# Autodesk Inventor assembly: Ensamble
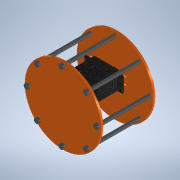
[picture p0: Inventor's stored thumbnail of the model, 180x180]
Saved by Autodesk Inventor 2021 (Build 250183000, 183)
## iProperties
Created: 2021-04-02
Part Number: Ensamble
Document SubType Name: Assembly
Designer: diego
Author: diego
## Documents named in this file (5)
- C:\Users\diego\Desktop\Diego\Utadeo 2021-1\Robotica Industrial\Corte 2\Solido planos\Ensamble.iam
- C:\Users\diego\Desktop\Diego\Utadeo 2021-1\Robotica Industrial\Corte 2\Solido planos\Base3.ipt
- C:\Users\diego\Desktop\Diego\Utadeo 2021-1\Robotica Industrial\Corte 2\Solido planos\Tornillo.ipt
- C:\Users\diego\Desktop\Diego\Utadeo 2021-1\Robotica Industrial\Corte 2\Solido planos\Servo.ipt
- C:\Users\diego\Desktop\Diego\Utadeo 2021-1\Robotica Industrial\Corte 2\Solido planos\Base1.iam
## Components (11 placed, 4 different names)
1. Base3:1 — Rígido:1, Rígido:2, Rígido:3, Rígido:4, Rígido:5, Rígido:6, Rígido:7, Rígido:8
2. Tornillo:1 — Rígido:1
3. Tornillo:2 — Rígido:2, Rígido:9
4. Tornillo:3 — Rígido:3
5. Tornillo:4 — Rígido:4
6. Tornillo:5 — Rígido:5
7. Tornillo:6 — Rígido:6
8. Tornillo:7 — Rígido:7
9. Tornillo:8 — Rígido:8
10. Servo:1 — Coincidencia:1
11. Base1:1 [sub-assembly] — Rígido:9, Coincidencia:1
## Relationships (10: WeldJoint 9, Mate 1)
- Rígido:1 [WeldJoint]: Base3:1 ↔ Tornillo:1
- Rígido:2 [WeldJoint]: Base3:1 ↔ Tornillo:2
- Rígido:3 [WeldJoint]: Base3:1 ↔ Tornillo:3
- Rígido:4 [WeldJoint]: Base3:1 ↔ Tornillo:4
- Rígido:5 [WeldJoint]: Base3:1 ↔ Tornillo:5
- Rígido:6 [WeldJoint]: Base3:1 ↔ Tornillo:6
- Rígido:7 [WeldJoint]: Base3:1 ↔ Tornillo:7
- Rígido:8 [WeldJoint]: Base3:1 ↔ Tornillo:8
- Rígido:9 [WeldJoint]: Tornillo:2 ↔ Base1:1
- Coincidencia:1 [Mate]: Servo:1 ↔ Base1:1
